# Autodesk Inventor assembly: Assembly2
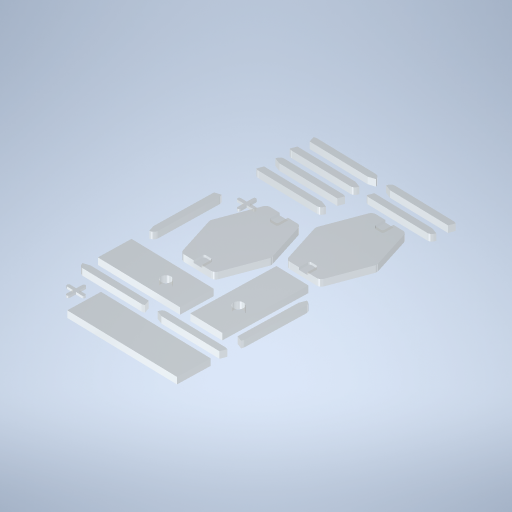
[picture p0: Inventor's stored thumbnail of the model, 512x512]
Saved by Autodesk Inventor 2024 (Build 280153000, 153)
## iProperties
Created: 2022-10-28
Part Number: Assembly2
Document SubType Name: Assembly
Designer: jshin23
Author: jshin23
## Documents named in this file (6)
- C:\Users\sjise\Documents\Kids Toy\Kids Toy\Assembly2.iam
- C:\Users\sjise\Documents\Kids Toy\Kids Toy\Part1 x 2.ipt
- C:\Users\sjise\Documents\Kids Toy\Kids Toy\Part3 x 2.ipt
- C:\Users\sjise\Documents\Kids Toy\Kids Toy\Part4 x 12.ipt
- C:\Users\sjise\Documents\Kids Toy\Kids Toy\Part2 x 1.ipt
- C:\Users\sjise\Documents\Kids Toy\Kids Toy\3DPart7 x 2.ipt
## Components (17 placed, 5 different names)
1. Part1 x 2:1 — Flush:3, Flush:5, Flush:6, Flush:7, Flush:8, Mate:3, Flush:22, Mate:27, Flush:23, Flush:24, Flush:25, Flush:28, Flush:36, Flush:38, Flush:40, Flush:41, Flush:42, Flush:43, Mate:35
2. Part1 x 2:2 — Mate:27, Flush:26, Flush:27, Flush:28, Flush:29, Flush:37
3. Part3 x 2:1 — Flush:3, Mate:3, Mate:4, Mate:15, Mate:19, Flush:27, Flush:34, Flush:35, Flush:36
4. Part3 x 2:2 — Mate:19, Mate:21, Flush:26, Flush:30
5. Part4 x 12:1 — Flush:5, Mate:4, Flush:18, Mate:16, Flush:19, Flush:35
6. Part4 x 12:2 — Flush:6, Flush:42, Flush:45, Mate:30, Mate:32
7. Part4 x 12:3 — Flush:7, Mate:14, Mate:15, Mate:16, Mate:17, Flush:20, Flush:33, Flush:34
8. Part4 x 12:4 — Flush:8, Flush:43, Mate:33, Mate:34
9. Part4 x 12:7 — Flush:29, Flush:37
10. Part4 x 12:9 — Mate:8, Mate:17, Mate:21, Flush:30, Flush:31
11. Part4 x 12:11 — Flush:41, Flush:45, Mate:30, Mate:31
12. Part2 x 1:1 — Mate:8, Flush:18, Mate:14, Flush:19, Mate:22, Flush:20, Flush:31, Flush:33, Flush:44
13. 3DPart7 x 2:1 — Mate:22, Flush:44
14. 3DPart7 x 2:2 — Flush:22
15. Part4 x 12:12 — Flush:23, Flush:38, Flush:39, Mate:31, Mate:33
16. Part4 x 12:13 — Flush:24, Flush:39, Mate:34
17. Part4 x 12:14 — Flush:25, Flush:40, Mate:32, Mate:35
## Relationships (48: Flush 31, Mate 17)
- Flush:3: Part1 x 2:1 ↔ Part3 x 2:1
- Flush:5: Part1 x 2:1 ↔ Part4 x 12:1
- Flush:6: Part1 x 2:1 ↔ Part4 x 12:2
- Flush:7: Part1 x 2:1 ↔ Part4 x 12:3
- Flush:8: Part1 x 2:1 ↔ Part4 x 12:4
- Mate:3 (20.32 mm): Part1 x 2:1 ↔ Part3 x 2:1
- Mate:4 (20.32 mm): Part3 x 2:1 ↔ Part4 x 12:1
- Mate:8 (20.32 mm): Part4 x 12:9 ↔ Part2 x 1:1
- Flush:18: Part4 x 12:1 ↔ Part2 x 1:1
- Mate:14 (20.32 mm): Part4 x 12:3 ↔ Part2 x 1:1
- Mate:15 (20.32 mm): Part3 x 2:1 ↔ Part4 x 12:3
- Mate:16: Part4 x 12:1 ↔ Part4 x 12:3
- Mate:17 (20.32 mm): Part4 x 12:3 ↔ Part4 x 12:9
- Mate:19 (20.32 mm): Part3 x 2:1 ↔ Part3 x 2:2
- Mate:21 (20.32 mm): Part3 x 2:2 ↔ Part4 x 12:9
- Flush:19: Part4 x 12:1 ↔ Part2 x 1:1
- Mate:22 (20.32 mm): Part2 x 1:1 ↔ 3DPart7 x 2:1
- Flush:20: Part4 x 12:3 ↔ Part2 x 1:1
- Flush:22: Part1 x 2:1 ↔ 3DPart7 x 2:2
- Mate:27 (20.32 mm): Part1 x 2:1 ↔ Part1 x 2:2
- Flush:23: Part1 x 2:1 ↔ Part4 x 12:12
- Flush:24: Part1 x 2:1 ↔ Part4 x 12:13
- Flush:25: Part1 x 2:1 ↔ Part4 x 12:14
- Flush:26: Part1 x 2:2 ↔ Part3 x 2:2
- Flush:27: Part1 x 2:2 ↔ Part3 x 2:1
- Flush:28: Part1 x 2:1 ↔ Part1 x 2:2
- Flush:29: Part1 x 2:2 ↔ Part4 x 12:7
- Flush:30: Part3 x 2:2 ↔ Part4 x 12:9
- Flush:31: Part4 x 12:9 ↔ Part2 x 1:1
- Flush:33: Part4 x 12:3 ↔ Part2 x 1:1
- Flush:34: Part3 x 2:1 ↔ Part4 x 12:3
- Flush:35: Part3 x 2:1 ↔ Part4 x 12:1
- Flush:36: Part1 x 2:1 ↔ Part3 x 2:1
- Flush:37: Part1 x 2:2 ↔ Part4 x 12:7
- Flush:38: Part1 x 2:1 ↔ Part4 x 12:12
- Flush:39: Part4 x 12:12 ↔ Part4 x 12:13
- Flush:40: Part1 x 2:1 ↔ Part4 x 12:14
- Flush:41: Part1 x 2:1 ↔ Part4 x 12:11
- Flush:42: Part1 x 2:1 ↔ Part4 x 12:2
- Flush:43: Part1 x 2:1 ↔ Part4 x 12:4
- Flush:44: Part2 x 1:1 ↔ 3DPart7 x 2:1
- Flush:45: Part4 x 12:2 ↔ Part4 x 12:11
- Mate:30 (20.32 mm): Part4 x 12:2 ↔ Part4 x 12:11
- Mate:31 (20.32 mm): Part4 x 12:11 ↔ Part4 x 12:12
- Mate:32 (20.32 mm): Part4 x 12:2 ↔ Part4 x 12:14
- Mate:33 (20.32 mm): Part4 x 12:4 ↔ Part4 x 12:12
- Mate:34 (20.32 mm): Part4 x 12:4 ↔ Part4 x 12:13
- Mate:35 (20.32 mm): Part1 x 2:1 ↔ Part4 x 12:14
